# Autodesk Inventor assembly: Cover V3 Assembly
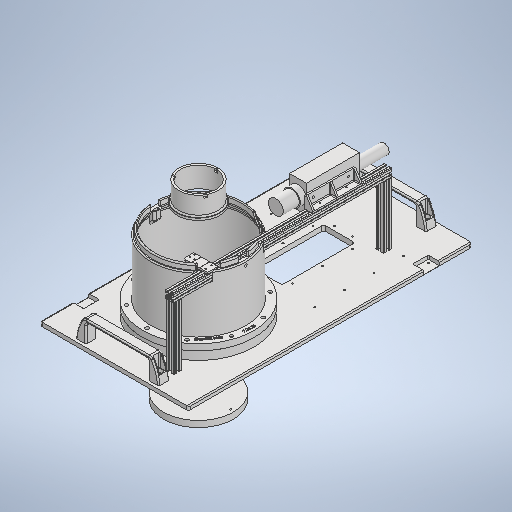
[picture p0: Inventor's stored thumbnail of the model, 512x512]
Saved by Autodesk Inventor 2025 (Build 290162000, 162)
## iProperties
Created: 2025-06-17
Part Number: Cover V3 Assembly
Document SubType Name: Assembly
Designer: mumin
Author: mumin
## Documents named in this file (15)
- C:\GitHub\In-situ-monitoring-of-powder-bed-fusion-additive-manufacturing\system_development\Orichalcum\v0.3\Cover v3 Assembly\Cover V3 Assembly.iam
- C:\GitHub\In-situ-monitoring-of-powder-bed-fusion-additive-manufacturing\system_development\Orichalcum\v0.3\Cover v3 Assembly\2020 Legs (150mm).ipt
- C:\GitHub\In-situ-monitoring-of-powder-bed-fusion-additive-manufacturing\system_development\Orichalcum\v0.3\Cover v3 Assembly\2020 LV-GVS Beam (530).ipt
- C:\GitHub\In-situ-monitoring-of-powder-bed-fusion-additive-manufacturing\system_development\Orichalcum\v0.3\Cover v3 Assembly\LV_Bracket_2.ipt
- C:\GitHub\In-situ-monitoring-of-powder-bed-fusion-additive-manufacturing\system_development\Orichalcum\v0.3\Cover v3 Assembly\12mm Cover.ipt
- C:\GitHub\In-situ-monitoring-of-powder-bed-fusion-additive-manufacturing\system_development\Orichalcum\v0.3\Cover v3 Assembly\Build Plate.ipt
- C:\GitHub\In-situ-monitoring-of-powder-bed-fusion-additive-manufacturing\system_development\Orichalcum\v0.3\Cover v3 Assembly\Updated Laser Scanner.ipt
- C:\GitHub\In-situ-monitoring-of-powder-bed-fusion-additive-manufacturing\system_development\Orichalcum\v0.3\Cover v3 Assembly\SealedGlassRing.ipt
- C:\GitHub\In-situ-monitoring-of-powder-bed-fusion-additive-manufacturing\system_development\Orichalcum\v0.3\Cover v3 Assembly\Cylinder Housing_base.ipt
- C:\GitHub\In-situ-monitoring-of-powder-bed-fusion-additive-manufacturing\system_development\Orichalcum\v0.3\Cover v3 Assembly\Cylinder Housing_Cap.ipt
- C:\GitHub\In-situ-monitoring-of-powder-bed-fusion-additive-manufacturing\system_development\Orichalcum\v0.3\Handle.ipt
- C:\GitHub\In-situ-monitoring-of-powder-bed-fusion-additive-manufacturing\system_development\Orichalcum\v0.3\Cover v3 Assembly\GVS_Plate.ipt
- C:\GitHub\In-situ-monitoring-of-powder-bed-fusion-additive-manufacturing\system_development\Orichalcum\v0.3\Cover v3 Assembly\Center Cylinder.ipt
- C:\GitHub\In-situ-monitoring-of-powder-bed-fusion-additive-manufacturing\system_development\Orichalcum\v0.3\Cover v3 Assembly\Cylinder-Plate Joiner.ipt
- C:\GitHub\In-situ-monitoring-of-powder-bed-fusion-additive-manufacturing\system_development\Orichalcum\v0.3\Cover v3 Assembly\Metal Head Plate.ipt
## Components (16 placed, 14 different names)
1. 12mm Cover:1 — Insert:4, Mate:4, Mate:5, Mate:6, Insert:11, Insert:12, Insert:15, Insert:16
2. Build Plate:1 — Insert:4
3. SealedGlassRing:1 — Mate:4, Insert:10
4. Cylinder Housing_base:1 — Insert:10, Mate:8
5. 2020 Legs (150mm):1 — Mate:5, Insert:11, Flush:1, Flush:2, Mate:7
6. 2020 Legs (150mm):2 — Mate:6, Insert:12, Flush:4
7. 2020 LV-GVS Beam (530):1 — Flush:1, Flush:2, Mate:7, Mate:9, Flush:3, Flush:4, Flush:5, Mate:10
8. Cylinder Housing_Cap:1 — Mate:8, Tangent:1
9. LV_Bracket_2:1 — Mate:9, Flush:3, Insert:13, Insert:14
10. Updated Laser Scanner:1 — Insert:13, Insert:14
11. Handle:1 — Insert:15
12. Handle:2 — Insert:16
13. GVS_Plate:1 — Flush:5, Mate:10
14. Center Cylinder:1 — Tangent:1, Insert:17
15. Cylinder-Plate Joiner:1 — Insert:17, Insert:18
16. Metal Head Plate:1 — Insert:18
## Relationships (23: Insert 10, Mate 7, Flush 5, Tangent 1)
- Insert:4 (150 mm): 12mm Cover:1 ↔ Build Plate:1
- Mate:4: 12mm Cover:1 ↔ SealedGlassRing:1
- Insert:10: SealedGlassRing:1 ↔ Cylinder Housing_base:1
- Mate:5: 12mm Cover:1 ↔ 2020 Legs (150mm):1
- Mate:6: 12mm Cover:1 ↔ 2020 Legs (150mm):2
- Insert:11: 12mm Cover:1 ↔ 2020 Legs (150mm):1
- Insert:12: 12mm Cover:1 ↔ 2020 Legs (150mm):2
- Flush:1: 2020 Legs (150mm):1 ↔ 2020 LV-GVS Beam (530):1
- Flush:2: 2020 Legs (150mm):1 ↔ 2020 LV-GVS Beam (530):1
- Mate:7: 2020 Legs (150mm):1 ↔ 2020 LV-GVS Beam (530):1
- Mate:8: Cylinder Housing_base:1 ↔ Cylinder Housing_Cap:1
- Mate:9: 2020 LV-GVS Beam (530):1 ↔ LV_Bracket_2:1
- Flush:3: 2020 LV-GVS Beam (530):1 ↔ LV_Bracket_2:1
- Flush:4: 2020 Legs (150mm):2 ↔ 2020 LV-GVS Beam (530):1
- Insert:13: LV_Bracket_2:1 ↔ Updated Laser Scanner:1
- Insert:14: LV_Bracket_2:1 ↔ Updated Laser Scanner:1
- Insert:15: 12mm Cover:1 ↔ Handle:1
- Insert:16: 12mm Cover:1 ↔ Handle:2
- Flush:5: 2020 LV-GVS Beam (530):1 ↔ GVS_Plate:1
- Mate:10: 2020 LV-GVS Beam (530):1 ↔ GVS_Plate:1
- Tangent:1: Cylinder Housing_Cap:1 ↔ Center Cylinder:1
- Insert:17: Center Cylinder:1 ↔ Cylinder-Plate Joiner:1
- Insert:18: Cylinder-Plate Joiner:1 ↔ Metal Head Plate:1
